# Autodesk Inventor assembly: 00_NEMA11
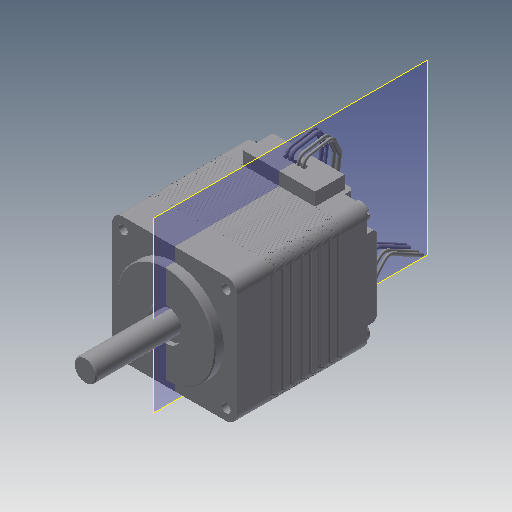
[picture p0: Inventor's stored thumbnail of the model, 512x512]
Saved by Autodesk Inventor 2019.4 (Build 234330000, 330)
## iProperties
Created: 2020-09-13
Part Number: 00_NEMA11
Description: STEP AP203
Document SubType Name: Assembly
Designer: diederichbenedict
Sending System: SolidWorks 2013
Preprocessor: SwSTEP 2.0
Title: NEMA11.STEP
Revision Number: ANY
## Documents named in this file (6)
- C:\Users\diederichbenedict\Dropbox\Dokumente\Promotion\PROJECTS\OPENTRONS\INVENTOR\00_NEMA11.iam
- C:\Users\diederichbenedict\Dropbox\Dokumente\Promotion\PROJECTS\OPENTRONS\INVENTOR\Opentrons_Rails\Workspace\Lagerschild_11.ipt
- C:\Users\diederichbenedict\Dropbox\Dokumente\Promotion\PROJECTS\OPENTRONS\INVENTOR\Opentrons_Rails\Workspace\Welle_11.ipt
- C:\Users\diederichbenedict\Dropbox\Dokumente\Promotion\PROJECTS\OPENTRONS\INVENTOR\Opentrons_Rails\Workspace\Kollektorschild_11.ipt
- C:\Users\diederichbenedict\Dropbox\Dokumente\Promotion\PROJECTS\OPENTRONS\INVENTOR\Opentrons_Rails\Workspace\Schraube_M2x25.ipt
- C:\Users\diederichbenedict\Dropbox\Dokumente\Promotion\PROJECTS\OPENTRONS\INVENTOR\Opentrons_Rails\Workspace\Stator_11.ipt
## Components (8 placed, 8 different names)
1. Lagerschild_11_1 — Symmetry:1
2. Welle_11_2
3. Kollektorschild_11_3 — Symmetry:1
4. Schraube_M2x25_4
5. Schraube_M2x25_5
6. Schraube_M2x25_6
7. Schraube_M2x25_7
8. Stator_11_8
## Relationships (1: Symmetry 1)
- Symmetry:1: Lagerschild_11_1 ↔ Kollektorschild_11_3
